# Autodesk Inventor assembly: ギアボックスv2
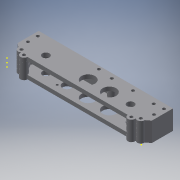
[picture p0: Inventor's stored thumbnail of the model, 180x180]
Saved by Autodesk Inventor 2018 (Build 220112000, 112)
## iProperties
Created: 2018-11-27
Part Number: ギアボックスv2
Material: 一般
Document SubType Name: Assembly
Designer: shun2
Author: shun2
## Documents named in this file (4)
- C:\Users\shun2\OneDrive\おそらく最新版(2018.7.31)\ギアボックス\ギアボックスv2.iam
- C:\Users\shun2\OneDrive\おそらく最新版(2018.7.31)\ギアボックス\1枚目\1枚目.ipt
- C:\Users\shun2\OneDrive\おそらく最新版(2018.7.31)\ギアボックス\2~4枚目\2-4枚目.ipt
- C:\Users\shun2\OneDrive\おそらく最新版(2018.7.31)\ギアボックス\5枚目\5枚目.ipt
## Components (5 placed, 3 different names)
1. 2-4枚目:1 — メイト:1, メイト:2, メイト:3, メイト:4, メイト:5, メイト:6
2. 2-4枚目:2 — メイト:4, メイト:5, メイト:6, メイト:7, メイト:8, メイト:9
3. 2-4枚目:3 — メイト:7, メイト:8, メイト:9, メイト:10, メイト:11, メイト:12
4. 1枚目:1 — メイト:1, メイト:2, メイト:3
5. 5枚目:1 — メイト:10, メイト:11, メイト:12
## Relationships (12: Mate 12)
- メイト:1 [Mate]: 2-4枚目:1 ↔ 1枚目:1
- メイト:2 [Mate]: 2-4枚目:1 ↔ 1枚目:1
- メイト:3 [Mate]: 2-4枚目:1 ↔ 1枚目:1
- メイト:4 [Mate]: 2-4枚目:1 ↔ 2-4枚目:2
- メイト:5 [Mate]: 2-4枚目:1 ↔ 2-4枚目:2
- メイト:6 [Mate]: 2-4枚目:1 ↔ 2-4枚目:2
- メイト:7 [Mate]: 2-4枚目:2 ↔ 2-4枚目:3
- メイト:8 [Mate]: 2-4枚目:2 ↔ 2-4枚目:3
- メイト:9 [Mate]: 2-4枚目:2 ↔ 2-4枚目:3
- メイト:10 [Mate]: 2-4枚目:3 ↔ 5枚目:1
- メイト:11 [Mate]: 2-4枚目:3 ↔ 5枚目:1
- メイト:12 [Mate]: 2-4枚目:3 ↔ 5枚目:1
